# Autodesk Inventor assembly: Assembly_Cube_Electric_Adpater
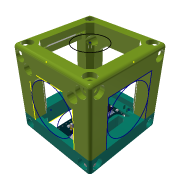
[picture p0: Inventor's stored thumbnail of the model, 180x180]
Saved by Autodesk Inventor 2019 (Build 230136000, 136)
## iProperties
Created: 2018-05-25
Part Number: Assembly_Cube_Electric_Adpater
Material: Generisch
Document SubType Name: Assembly
Designer: diederichbenedict
Mass: 12.1987 g
Surface Area: 115.22 cm^2
Volume: 11.001 cm^3
Density: 1.10887 g/cm^3
Author: diederichbenedict
## Documents named in this file (5)
- C:\Users\diederichbenedict\Dropbox\Dokumente\Promotion\PROJECTS\UC2\01-Fluidicscope\02_CAD\INVENTOR\E.ColiV4\10_Cube_Base\Assembly_Cube_Electric_Adpater.iam
- C:\Users\diederichbenedict\Dropbox\Dokumente\Promotion\PROJECTS\UC2\01-Fluidicscope\02_CAD\INVENTOR\E.ColiV4\10_Cube_Base\10_Lid_el_v0.ipt
- C:\Users\diederichbenedict\Dropbox\Dokumente\Promotion\PROJECTS\UC2\01-Fluidicscope\02_CAD\INVENTOR\E.ColiV4\10_Cube_Base\arduino nano.ipt
- C:\Users\diederichbenedict\Dropbox\Dokumente\Promotion\PROJECTS\UC2\01-Fluidicscope\02_CAD\INVENTOR\E.ColiV4\CONFOCAL_Haoran\DIN 912 - M3 x 0,5 x 12 x 10,75.ipt
- C:\Users\diederichbenedict\Dropbox\Dokumente\Promotion\PROJECTS\UC2\01-Fluidicscope\02_CAD\INVENTOR\E.ColiV4\10_Cube_Base\10_Cube_v0.ipt
## Components (7 placed, 4 different names)
1. 10_Lid_el_v0:1 — Fluchtend:1, Fluchtend:2, Fluchtend:3, Einfügen:1, Mate:1, Flush:4, Flush:5, Insert:2, Insert:3, Insert:4
2. arduino nano:1 — Fluchtend:1, Fluchtend:2, Fluchtend:3
3. DIN 912 - ersetzt durch DIN EN ISO 4762 M3 x 12:1 — Einfügen:1
4. 10_Cube_v0:1 — Mate:1, Flush:4, Flush:5
5. DIN 912 - ersetzt durch DIN EN ISO 4762 M3 x 12:2 — Insert:4
6. DIN 912 - ersetzt durch DIN EN ISO 4762 M3 x 12:3 — Insert:2
7. DIN 912 - ersetzt durch DIN EN ISO 4762 M3 x 12:4 — Insert:3
## Relationships (10: Flush 5, Insert 4, Mate 1)
- Fluchtend:1 [Flush] (16 mm): 10_Lid_el_v0:1 ↔ arduino nano:1
- Fluchtend:2 [Flush]: 10_Lid_el_v0:1 ↔ arduino nano:1
- Fluchtend:3 [Flush] (3 mm): 10_Lid_el_v0:1 ↔ arduino nano:1
- Einfügen:1 [Insert]: 10_Lid_el_v0:1 ↔ DIN 912 - ersetzt durch DIN EN ISO 4762 M3 x 12:1
- Mate:1: 10_Lid_el_v0:1 ↔ 10_Cube_v0:1
- Flush:4: 10_Lid_el_v0:1 ↔ 10_Cube_v0:1
- Flush:5: 10_Lid_el_v0:1 ↔ 10_Cube_v0:1
- Insert:2: 10_Lid_el_v0:1 ↔ DIN 912 - ersetzt durch DIN EN ISO 4762 M3 x 12:3
- Insert:3: 10_Lid_el_v0:1 ↔ DIN 912 - ersetzt durch DIN EN ISO 4762 M3 x 12:4
- Insert:4: 10_Lid_el_v0:1 ↔ DIN 912 - ersetzt durch DIN EN ISO 4762 M3 x 12:2
